# Autodesk Inventor assembly: Belt_Holder
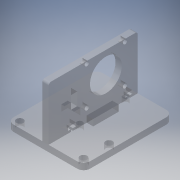
[picture p0: Inventor's stored thumbnail of the model, 180x180]
Saved by Autodesk Inventor 2016 (Build 200138000, 138)
## iProperties
Created: 2018-05-31
Part Number: Belt_Holder
Document SubType Name: Assembly
Designer: Phil Erle
Author: Phil Erle
## Documents named in this file (3)
- C:\Users\Phil Erle\Desktop\Adrastea\Belt_Holder.iam
- C:\Users\Phil Erle\Desktop\Adrastea\Belt_Holder1.ipt
- C:\Users\Phil Erle\Desktop\Adrastea\Belt_Holder2.ipt
## Components (2 placed, 2 different names)
1. Belt_Holder1:1 — Flush:1, Flush:2, Flush:3, Mate:1, Mate:2, Mate:3
2. Belt_Holder2:1 — Mate:1, Mate:2, Mate:3
## Relationships (6: Flush 3, Mate 3)
- Flush:1: Belt_Holder1:1
- Flush:2: Belt_Holder1:1
- Flush:3: Belt_Holder1:1
- Mate:1: Belt_Holder1:1 ↔ Belt_Holder2:1
- Mate:2: Belt_Holder1:1 ↔ Belt_Holder2:1
- Mate:3: Belt_Holder1:1 ↔ Belt_Holder2:1
